# Autodesk Inventor assembly: am14u3LongWithSlideMechanism
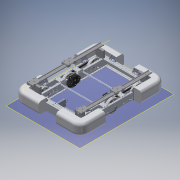
[picture p0: Inventor's stored thumbnail of the model, 180x180]
Saved by Autodesk Inventor 2018.2 (Build 222227000, 227)
## iProperties
Created: 2018-01-15
Part Number: am14u3LongWithSlideMechanism
Document SubType Name: Assembly
Designer: steele
Author: steele
## Documents named in this file (11)
- D:\snobotics\CAD-Development\robSteele\2018-FRC\am14u3LongWithSlideMechanism.iam
- D:\snobotics\CAD-Development\robSteele\2018-FRC\AMbaseLongWithBumper\Long with Bumper\DB_DriveBaseLong_AM14U3_Bumpers and Battery Tray.iam
- D:\snobotics\CAD-Development\robSteele\2018-FRC\Rail System\6109K422 rail 33 inches long.ipt
- D:\snobotics\CAD-Development\robSteele\2018-FRC\Rail System\supportBlock.ipt
- D:\snobotics\CAD-Development\robSteele\2018-FRC\Rail System\supportBlock_MIR.ipt
- D:\snobotics\CAD-Development\robSteele\2018-FRC\Rail System\supportBlock_MIR1.ipt
- D:\snobotics\CAD-Development\robSteele\2018-FRC\Rail System\supportBlock_MIR_MIR.ipt
- D:\snobotics\CAD-Development\robSteele\2018-FRC\Rail System\6109K422 rail 33 inches long_MIR.ipt
- D:\snobotics\CAD-Development\robSteele\2018-FRC\Rail System\6109K410 carriage.ipt
- D:\snobotics\CAD-Development\robSteele\2018-FRC\Rail System\6109K410 carriage_MIR.ipt
- D:\snobotics\CAD-Development\robSteele\2018-FRC\Rail System\6109K410 carriage_MIR1.ipt
## Components (11 placed, 10 different names)
1. DB_DriveBaseLong_AM14U3_Bumpers and Battery Tray:1 [sub-assembly] — Flush:2, Flush:3, Mate:1, Mate:2, Mate:4, Flush:4
2. 6109K422 rail 33 inches long:1 — Mate:3, Mate:4, Flush:4, Insert:1, Insert:2, Insert:3, Insert:4
3. supportBlock:1 — Flush:3, Mate:1, Mate:2, Mate:3
4. supportBlock_MIR:1
5. supportBlock_MIR1:1
6. supportBlock_MIR_MIR:1
7. 6109K422 rail 33 inches long_MIR:1
8. 6109K410 carriage:1 — Insert:1, Insert:2
9. 6109K410 carriage_MIR:1
10. 6109K410 carriage:2 — Insert:3, Insert:4
11. 6109K410 carriage_MIR1:1
## Relationships (11: Mate 4, Insert 4, Flush 3)
- Flush:2 (50.8 mm): DB_DriveBaseLong_AM14U3_Bumpers and Battery Tray:1
- Flush:3: DB_DriveBaseLong_AM14U3_Bumpers and Battery Tray:1 ↔ supportBlock:1
- Mate:1: DB_DriveBaseLong_AM14U3_Bumpers and Battery Tray:1 ↔ supportBlock:1
- Mate:2: DB_DriveBaseLong_AM14U3_Bumpers and Battery Tray:1 ↔ supportBlock:1
- Mate:3: 6109K422 rail 33 inches long:1 ↔ supportBlock:1
- Mate:4: DB_DriveBaseLong_AM14U3_Bumpers and Battery Tray:1 ↔ 6109K422 rail 33 inches long:1
- Flush:4: DB_DriveBaseLong_AM14U3_Bumpers and Battery Tray:1 ↔ 6109K422 rail 33 inches long:1
- Insert:1 (406.4 mm): 6109K422 rail 33 inches long:1 ↔ 6109K410 carriage:1
- Insert:2 (406.4 mm): 6109K422 rail 33 inches long:1 ↔ 6109K410 carriage:1
- Insert:3: 6109K422 rail 33 inches long:1 ↔ 6109K410 carriage:2
- Insert:4: 6109K422 rail 33 inches long:1 ↔ 6109K410 carriage:2
## Named parameters: carriageDistanceFromEnd = 406.4 mm
